# Autodesk Inventor assembly: Assembly1
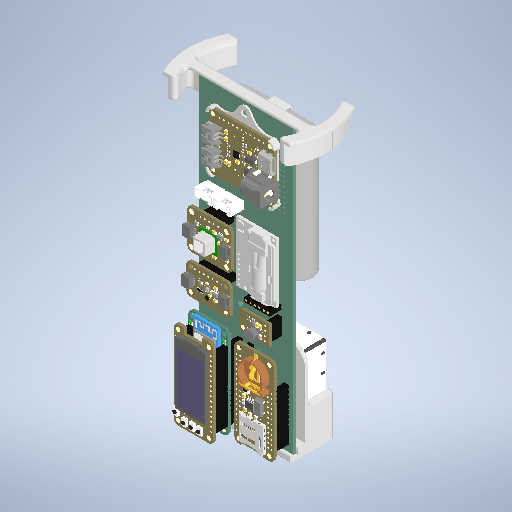
[picture p0: Inventor's stored thumbnail of the model, 512x512]
Saved by Autodesk Inventor 2025.3 (Build 293356000, 356)
## iProperties
Created: 2024-07-03
Part Number: Assembly1
Document SubType Name: Assembly
Designer: vncnt
Author: vncnt
## Documents named in this file (21)
- C:\Users\vncnt\OneDrive\Documents\Inventor\ASRC\Air Quality Sensor\Air Quality Sensor\AQS Assembly.iam
- C:\Users\vncnt\OneDrive\Documents\Inventor\ASRC\Air Quality Sensor\Air Quality Board Mount\PVC.ipt
- C:\Users\vncnt\OneDrive\Documents\Inventor\ASRC\Air Quality Sensor\Air Quality Board Mount\CSL AQS V1 spin3.iam
- C:\Users\vncnt\OneDrive\Documents\Inventor\ASRC\Air Quality Sensor\Air Quality Board Mount\AQS Mount V6.ipt
- C:\Users\vncnt\OneDrive\Documents\Inventor\ASRC\Air Quality Sensor\Air Quality Sensor\Sensirion STEP SEN5x\Sensirion STEP SEN5x.ipt
- C:\Users\vncnt\OneDrive\Documents\Inventor\ASRC\Air Quality Sensor\Air Quality Board Mount\SEN5X Mount V4.ipt
- C:\Users\vncnt\OneDrive\Documents\Inventor\ASRC\Air Quality Sensor\Air Quality Sensor\head_f_4p.ipt
- C:\Users\vncnt\OneDrive\Documents\Inventor\ASRC\Air Quality Sensor\Air Quality Sensor\3010 Adafruit Feather M0 WiFi\3010 Adafruit Feather M0 WiFi\3010 Adafruit Feather M0 WiFi.ipt
- C:\Users\vncnt\OneDrive\Documents\Inventor\ASRC\Air Quality Sensor\Air Quality Sensor\4650 OLED FeatherWing.ipt
- C:\Users\vncnt\OneDrive\Documents\Inventor\ASRC\Air Quality Sensor\Air Quality Sensor\head_f_3p.ipt
- C:\Users\vncnt\OneDrive\Documents\Inventor\ASRC\Air Quality Sensor\Air Quality Sensor\head_f_2p.ipt
- C:\Users\vncnt\OneDrive\Documents\Inventor\ASRC\Air Quality Sensor\Air Quality Sensor\2652 BMP280 STEMMA QT.ipt
- C:\Users\vncnt\OneDrive\Documents\Inventor\ASRC\Air Quality Sensor\Air Quality Sensor\4654 MiniBoost 5V.ipt
- C:\Users\vncnt\OneDrive\Documents\Inventor\ASRC\Air Quality Sensor\Air Quality Sensor\5187 SCD-40 C02 Sensor.ipt
- C:\Users\vncnt\OneDrive\Documents\Inventor\ASRC\Air Quality Sensor\Air Quality Sensor\Sensirion_CO2_Sensors_SCD30_POD_STEP_File.ipt
- C:\Users\vncnt\OneDrive\Documents\Inventor\ASRC\Air Quality Sensor\Air Quality Sensor\Grove socket.ipt
- C:\Users\vncnt\OneDrive\Documents\Inventor\ASRC\Air Quality Sensor\Air Quality Sensor\2922 FeatherWing Adalogger.ipt
- C:\Users\vncnt\OneDrive\Documents\Inventor\ASRC\Air Quality Sensor\Air Quality Sensor\Solar Board Mount V1.ipt
- C:\Users\vncnt\OneDrive\Documents\Inventor\ASRC\Air Quality Sensor\Air Quality Sensor\4755 USB Solar Charger.iam
- C:\Users\vncnt\OneDrive\Documents\Inventor\ASRC\Air Quality Sensor\Air Quality Sensor\353 6600mAh Battery.ipt
- C:\Users\vncnt\OneDrive\Documents\Inventor\ASRC\Air Quality Sensor\Air Quality Sensor\Battery Mount V1.ipt
## Components (54 placed, 20 different names)
1. PVC:1 — Mate:1, Mate:2, Flush:1, Mate:5, Flush:2, Mate:16
2. Sensirion STEP SEN5x:1 — Mate:12, Mate:13, Mate:68
3. CSL AQS V1 spin3:1 [sub-assembly] — Mate:5, Mate:7, Mate:9, Mate:11, Mate:15, Mate:17, Mate:18, Mate:19, Mate:20, Mate:36, Mate:37, Mate:38, Mate:39, Mate:40, Mate:41, Mate:42, Mate:43, Mate:44, Mate:45, Mate:46, Mate:47, Mate:48, Mate:49, Mate:50, Mate:51, Mate:52, Mate:53, Mate:54, Mate:55, Mate:56, Mate:57, Mate:58, Mate:72, Mate:73, Mate:74, Mate:78, Mate:79, Mate:80, Mate:81, Mate:82, Mate:83, Mate:84, Mate:85, Mate:86, Mate:90, Mate:91, Mate:95, Angle:1
4. AQS Mount V6:1 — Mate:7, Flush:2, Mate:15, Mate:16, Mate:75, Mate:76, Mate:96
5. SEN5X Mount V4:1 — Mate:9, Mate:11, Mate:12, Mate:13, Mate:17, Mate:68, Mate:97
6. 3010 Adafruit Feather M0 WiFi:1 — Mate:27, Mate:28, Mate:29
7. 4650 OLED FeatherWing:1 — Mate:35
8. head_f_4p:39 — Mate:46, Mate:47, Mate:48, Flush:6
9. head_f_4p:41 — Mate:36, Mate:37, Mate:38, Flush:3, Mate:59
10. head_f_4p:42 — Mate:41, Mate:42, Mate:43, Flush:4, Mate:70
11. head_f_4p:43 — Mate:49, Mate:50, Mate:51, Mate:62, Mate:63, Mate:64
12. head_f_3p:1 — Mate:39, Mate:40, Flush:3, Mate:60, Mate:61
13. head_f_3p:2 — Mate:44, Mate:45, Flush:4, Mate:69, Mate:71
14. head_f_3p:3 — Mate:52, Mate:53, Mate:58, Flush:5, Mate:66
15. head_f_2p:1 — Mate:54, Mate:55, Flush:5, Mate:65, Mate:67
16. head_f_2p:2 — Mate:56, Mate:57, Flush:6
17. 2652 BMP280 STEMMA QT:1 — Mate:59, Mate:60, Mate:61
18. 4654 MiniBoost 5V:1 — Mate:62, Mate:63, Mate:64
19. 5187 SCD-40 C02 Sensor:1 — Mate:65, Mate:66, Mate:67
20. Sensirion_CO2_Sensors_SCD30_POD_STEP_File:1 — Mate:69, Mate:70, Mate:71
21. Grove socket:1 — Mate:73, Mate:76, Mate:77
22. Grove socket:2 — Mate:72, Mate:74, Mate:75, Mate:77
23. 2922 FeatherWing Adalogger:1 — Mate:87, Mate:88, Mate:89
24. Solar Board Mount V1:1 — Mate:90, Mate:91, Mate:92, Mate:93, Mate:94, Mate:95
25. 4755 USB Solar Charger:2 [sub-assembly] — Mate:92, Mate:93, Mate:94
26. 353 6600mAh Battery:1 — Mate:98, Mate:99, Flush:7
27. Battery Mount V1:1 — Mate:96, Mate:97, Angle:1, Mate:98, Mate:99, Flush:7
28. head_f_4p:2
29. head_f_4p:1 — Mate:18, Mate:19, Mate:20, Mate:27, Mate:29
30. head_f_4p:9
31. head_f_4p:10 — Mate:35
32. head_f_4p:11
33. head_f_4p:12 — Mate:28
34. head_f_4p:22
35. head_f_4p:23
36. head_f_4p:24
37. head_f_4p:25
38. head_f_4p:26
39. head_f_4p:27
40. head_f_4p:44 — Mate:78, Mate:79, Mate:80
41. head_f_4p:45
42. head_f_4p:46
43. head_f_4p:47
44. head_f_4p:48
45. head_f_4p:49
46. head_f_4p:50
47. head_f_4p:51
48. head_f_4p:52 — Mate:81, Mate:82, Mate:83, Mate:87
49. head_f_4p:54
50. head_f_4p:55
51. head_f_4p:56
52. head_f_4p:53 — Mate:84, Mate:85, Mate:86
53. head_f_4p:57 — Mate:89
54. head_f_4p:58 — Mate:88
## Component patterns: (6 elements, first: head_f_4p:2 + head_f_4p:1), (8 elements, first: head_f_4p:44), (4 elements, first: head_f_4p:52), (3 elements, first: head_f_4p:53)
## Relationships (90: Mate 82, Flush 7, Angle 1)
- Mate:1: PVC:1
- Mate:2: PVC:1
- Flush:1: PVC:1
- Mate:5: PVC:1 ↔ CSL AQS V1 spin3:1
- Mate:7: CSL AQS V1 spin3:1 ↔ AQS Mount V6:1
- Flush:2: PVC:1 ↔ AQS Mount V6:1
- Mate:9: CSL AQS V1 spin3:1 ↔ SEN5X Mount V4:1
- Mate:11: CSL AQS V1 spin3:1 ↔ SEN5X Mount V4:1
- Mate:12: Sensirion STEP SEN5x:1 ↔ SEN5X Mount V4:1
- Mate:13: Sensirion STEP SEN5x:1 ↔ SEN5X Mount V4:1
- Mate:15: CSL AQS V1 spin3:1 ↔ AQS Mount V6:1
- Mate:16: PVC:1 ↔ AQS Mount V6:1
- Mate:17: CSL AQS V1 spin3:1 ↔ SEN5X Mount V4:1
- Mate:18: CSL AQS V1 spin3:1 ↔ head_f_4p:1
- Mate:19: CSL AQS V1 spin3:1 ↔ head_f_4p:1
- Mate:20: CSL AQS V1 spin3:1 ↔ head_f_4p:1
- Mate:27: 3010 Adafruit Feather M0 WiFi:1 ↔ head_f_4p:1
- Mate:28: 3010 Adafruit Feather M0 WiFi:1 ↔ head_f_4p:12
- Mate:29: 3010 Adafruit Feather M0 WiFi:1 ↔ head_f_4p:1
- Mate:35: 4650 OLED FeatherWing:1 ↔ head_f_4p:10
- Mate:36: CSL AQS V1 spin3:1 ↔ head_f_4p:41
- Mate:37: CSL AQS V1 spin3:1 ↔ head_f_4p:41
- Mate:38: CSL AQS V1 spin3:1 ↔ head_f_4p:41
- Mate:39: CSL AQS V1 spin3:1 ↔ head_f_3p:1
- Mate:40: CSL AQS V1 spin3:1 ↔ head_f_3p:1
- Flush:3: head_f_4p:41 ↔ head_f_3p:1
- Mate:41: CSL AQS V1 spin3:1 ↔ head_f_4p:42
- Mate:42: CSL AQS V1 spin3:1 ↔ head_f_4p:42
- Mate:43: CSL AQS V1 spin3:1 ↔ head_f_4p:42
- Mate:44: CSL AQS V1 spin3:1 ↔ head_f_3p:2
- Mate:45: CSL AQS V1 spin3:1 ↔ head_f_3p:2
- Flush:4: head_f_4p:42 ↔ head_f_3p:2
- Mate:46: CSL AQS V1 spin3:1 ↔ head_f_4p:39
- Mate:47: CSL AQS V1 spin3:1 ↔ head_f_4p:39
- Mate:48: CSL AQS V1 spin3:1 ↔ head_f_4p:39
- Mate:49: CSL AQS V1 spin3:1 ↔ head_f_4p:43
- Mate:50: CSL AQS V1 spin3:1 ↔ head_f_4p:43
- Mate:51: CSL AQS V1 spin3:1 ↔ head_f_4p:43
- Mate:52: CSL AQS V1 spin3:1 ↔ head_f_3p:3
- Mate:53: CSL AQS V1 spin3:1 ↔ head_f_3p:3
- Mate:54: CSL AQS V1 spin3:1 ↔ head_f_2p:1
- Mate:55: CSL AQS V1 spin3:1 ↔ head_f_2p:1
- Mate:56: CSL AQS V1 spin3:1 ↔ head_f_2p:2
- Mate:57: CSL AQS V1 spin3:1 ↔ head_f_2p:2
- Mate:58: CSL AQS V1 spin3:1 ↔ head_f_3p:3
- Flush:5: head_f_3p:3 ↔ head_f_2p:1
- Flush:6: head_f_4p:39 ↔ head_f_2p:2
- Mate:59: head_f_4p:41 ↔ 2652 BMP280 STEMMA QT:1
- Mate:60: head_f_3p:1 ↔ 2652 BMP280 STEMMA QT:1
- Mate:61: head_f_3p:1 ↔ 2652 BMP280 STEMMA QT:1
- Mate:62: head_f_4p:43 ↔ 4654 MiniBoost 5V:1
- Mate:63: head_f_4p:43 ↔ 4654 MiniBoost 5V:1
- Mate:64: head_f_4p:43 ↔ 4654 MiniBoost 5V:1
- Mate:65: head_f_2p:1 ↔ 5187 SCD-40 C02 Sensor:1
- Mate:66: head_f_3p:3 ↔ 5187 SCD-40 C02 Sensor:1
- Mate:67: head_f_2p:1 ↔ 5187 SCD-40 C02 Sensor:1
- Mate:68: Sensirion STEP SEN5x:1 ↔ SEN5X Mount V4:1
- Mate:69: head_f_3p:2 ↔ Sensirion_CO2_Sensors_SCD30_POD_STEP_File:1
- Mate:70: head_f_4p:42 ↔ Sensirion_CO2_Sensors_SCD30_POD_STEP_File:1
- Mate:71: head_f_3p:2 ↔ Sensirion_CO2_Sensors_SCD30_POD_STEP_File:1
- Mate:72: CSL AQS V1 spin3:1 ↔ Grove socket:2
- Mate:73: CSL AQS V1 spin3:1 ↔ Grove socket:1
- Mate:74 (-15.4432 mm): CSL AQS V1 spin3:1 ↔ Grove socket:2
- Mate:75 (51.3461 mm): AQS Mount V6:1 ↔ Grove socket:2
- Mate:76 (51.3461 mm): AQS Mount V6:1 ↔ Grove socket:1
- Mate:77 (0.7112 mm): Grove socket:1 ↔ Grove socket:2
- Mate:78: CSL AQS V1 spin3:1 ↔ head_f_4p:44
- Mate:79: CSL AQS V1 spin3:1 ↔ head_f_4p:44
- Mate:80: CSL AQS V1 spin3:1 ↔ head_f_4p:44
- Mate:81: CSL AQS V1 spin3:1 ↔ head_f_4p:52
- Mate:82: CSL AQS V1 spin3:1 ↔ head_f_4p:52
- Mate:83: CSL AQS V1 spin3:1 ↔ head_f_4p:52
- Mate:84: CSL AQS V1 spin3:1 ↔ head_f_4p:53
- Mate:85: CSL AQS V1 spin3:1 ↔ head_f_4p:53
- Mate:86: CSL AQS V1 spin3:1 ↔ head_f_4p:53
- Mate:87: 2922 FeatherWing Adalogger:1 ↔ head_f_4p:52
- Mate:88: 2922 FeatherWing Adalogger:1 ↔ head_f_4p:58
- Mate:89: 2922 FeatherWing Adalogger:1 ↔ head_f_4p:57
- Mate:90: CSL AQS V1 spin3:1 ↔ Solar Board Mount V1:1
- Mate:91: CSL AQS V1 spin3:1 ↔ Solar Board Mount V1:1
- Mate:92: Solar Board Mount V1:1 ↔ 4755 USB Solar Charger:2
- Mate:93: Solar Board Mount V1:1 ↔ 4755 USB Solar Charger:2
- Mate:94: Solar Board Mount V1:1 ↔ 4755 USB Solar Charger:2
- Mate:95: CSL AQS V1 spin3:1 ↔ Solar Board Mount V1:1
- Mate:96: AQS Mount V6:1 ↔ Battery Mount V1:1
- Mate:97: SEN5X Mount V4:1 ↔ Battery Mount V1:1
- Angle:1 (90 deg): CSL AQS V1 spin3:1 ↔ Battery Mount V1:1
- Mate:98: 353 6600mAh Battery:1 ↔ Battery Mount V1:1
- Mate:99: 353 6600mAh Battery:1 ↔ Battery Mount V1:1
- Flush:7 (21.59 mm): 353 6600mAh Battery:1 ↔ Battery Mount V1:1
